# Autodesk Inventor assembly: CP2x1 test assembly
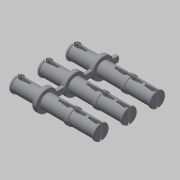
[picture p0: Inventor's stored thumbnail of the model, 180x180]
Saved by Autodesk Inventor 2019.3 (Build 233278000, 278)
## iProperties
Created: 2019-02-28
Part Number: CP2x1 test assembly
Document SubType Name: Assembly
Designer: Varga Daniel
Author: Varga Daniel
## Documents named in this file (6)
- C:\!_Dani\!_cloud\OneDrive\!_munka\Revolution\RevvyDemoKit\Structural parts\RFQ\SLS print collection Rev 1\CP2x1\CP2x1 test assembly.iam
- C:\!_Dani\!_cloud\OneDrive\!_munka\Revolution\RevvyDemoKit\Structural parts\RFQ\SLS print collection Rev 1\CP2x1\CP2x1_4,900_8,500_5,45.ipt
- C:\!_Dani\!_cloud\OneDrive\!_munka\Revolution\RevvyDemoKit\Structural parts\RFQ\SLS print collection Rev 1\CP2x1.ipt
- C:\!_Dani\!_cloud\OneDrive\!_munka\Revolution\RevvyDemoKit\Structural parts\RFQ\SLS print collection Rev 1\CP2x1\CP2x1_4,900_8,500_5,50.ipt
- C:\!_Dani\!_cloud\OneDrive\!_munka\Revolution\RevvyDemoKit\Structural parts\RFQ\SLS print collection Rev 1\CP2x1\CP2x1_4,900_8,500_5,55.ipt
- C:\!_Dani\!_cloud\OneDrive\!_munka\Revolution\RevvyDemoKit\Structural parts\RFQ\SLS print collection Rev 1\CP2x1\pin_interconnect_2.ipt
## Components (4 placed, 4 different names)
1. CP2x1_4,900_8,500_5,45:1 — Flush:1, Tangent:1, Flush:3, Flush:5, Mate:1
2. CP2x1_4,900_8,500_5,50:2 — Flush:1, Flush:2, Tangent:2, Flush:3, Flush:4
3. CP2x1_4,900_8,500_5,55:3 — Flush:2, Tangent:3, Flush:4
4. pin_interconnect_2:1 — Flush:5, Angle:1, Mate:1
## Relationships (10: Flush 5, Tangent 3, Angle 1, Mate 1)
- Flush:1: CP2x1_4,900_8,500_5,45:1 ↔ CP2x1_4,900_8,500_5,50:2
- Flush:2: CP2x1_4,900_8,500_5,50:2 ↔ CP2x1_4,900_8,500_5,55:3
- Tangent:1: CP2x1_4,900_8,500_5,45:1
- Tangent:2: CP2x1_4,900_8,500_5,50:2
- Tangent:3: CP2x1_4,900_8,500_5,55:3
- Flush:3 (-10 mm): CP2x1_4,900_8,500_5,45:1 ↔ CP2x1_4,900_8,500_5,50:2
- Flush:4 (-10 mm): CP2x1_4,900_8,500_5,50:2 ↔ CP2x1_4,900_8,500_5,55:3
- Flush:5 (0.3 mm): CP2x1_4,900_8,500_5,45:1 ↔ pin_interconnect_2:1
- Angle:1 (0 deg): pin_interconnect_2:1
- Mate:1: CP2x1_4,900_8,500_5,45:1 ↔ pin_interconnect_2:1
